# Autodesk Inventor assembly: Main
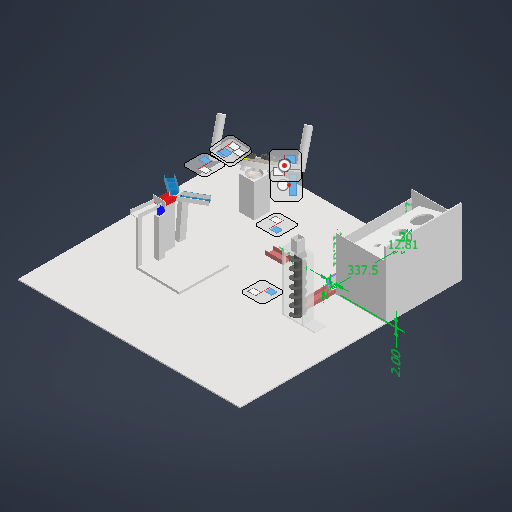
[picture p0: Inventor's stored thumbnail of the model, 512x512]
Saved by Autodesk Inventor 2026.2 (Build 302298000, 298)
## iProperties
Created: 2026-03-06
Part Number: Main
Document SubType Name: Assembly
Designer: danda
Author: danda
## Documents named in this file (8)
- C:\Users\danda\OneDrive\Desktop\Basics Of Mecha\Project\Main.iam
- C:\Users\danda\OneDrive\Desktop\Basics Of Mecha\Project\baseb.ipt
- C:\Users\danda\OneDrive\Desktop\Basics Of Mecha\Project\sorting\Assembly2.iam
- C:\Users\danda\OneDrive\Desktop\Basics Of Mecha\Project\Lifting\Assembly2.iam
- C:\Users\danda\OneDrive\Desktop\Basics Of Mecha\Project\Shooting Mechanism CAD\Shooting Mechanism Assembly.iam
- C:\Users\danda\OneDrive\Desktop\Basics Of Mecha\Project\collectingbox.ipt
- C:\Users\danda\OneDrive\Desktop\Basics Of Mecha\Project\5mmhieght.ipt
- C:\Users\danda\OneDrive\Desktop\Basics Of Mecha\Project\collectingslide.ipt
## Components (7 placed, 6 different names)
1. baseb:1 — Mate:1, Mate:2, Mate:3, Flush:1, Mate:6, Mate:7, Mate:9, Mate:11, Mate:14, Flush:5, Flush:6
2. Shooting Mechanism Assembly:1 [sub-assembly] — Mate:14, Flush:6
3. Assembly2:3 [sub-assembly] — Mate:6
4. Assembly2:4 [sub-assembly] — Mate:7, Mate:8, Mate:13, Flush:4
5. collectingbox:1 — Flush:1, Mate:8, Mate:10, Flush:2, Flush:3, Flush:5
6. 5mmhieght:1 — Mate:9, Mate:10, Flush:2, Flush:3, Mate:12
7. collectingslide:1 — Mate:11, Mate:12, Mate:13, Flush:4
## Relationships (18: Mate 12, Flush 6)
- Mate:1: baseb:1
- Mate:2: baseb:1
- Mate:3: baseb:1
- Flush:1: baseb:1 ↔ collectingbox:1
- Mate:6: baseb:1 ↔ Assembly2:3
- Mate:7: baseb:1 ↔ Assembly2:4
- Mate:8: Assembly2:4 ↔ collectingbox:1
- Mate:9: baseb:1 ↔ 5mmhieght:1
- Mate:10: collectingbox:1 ↔ 5mmhieght:1
- Flush:2: collectingbox:1 ↔ 5mmhieght:1
- Flush:3: collectingbox:1 ↔ 5mmhieght:1
- Mate:11: baseb:1 ↔ collectingslide:1
- Mate:12: 5mmhieght:1 ↔ collectingslide:1
- Mate:13: Assembly2:4 ↔ collectingslide:1
- Flush:4: Assembly2:4 ↔ collectingslide:1
- Mate:14: baseb:1 ↔ Shooting Mechanism Assembly:1
- Flush:5: baseb:1 ↔ collectingbox:1
- Flush:6 (170 mm): baseb:1 ↔ Shooting Mechanism Assembly:1
